# Autodesk Inventor assembly: Full Wheel
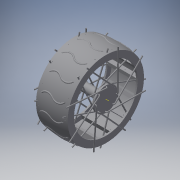
[picture p0: Inventor's stored thumbnail of the model, 180x180]
Saved by Autodesk Inventor 2019 (Build 230136000, 136)
## iProperties
Created: 2018-10-28
Part Number: Full Wheel
Document SubType Name: Assembly
Designer: Swapnil
Author: Swapnil
## Documents named in this file (3)
- C:\Users\Swapnil\Desktop\ImportantThings\Robotics\Vanderbilt Robotics\2018-2019\FrameAndDrive\Full Wheel.iam
- C:\Users\Swapnil\Desktop\ImportantThings\Robotics\Vanderbilt Robotics\2018-2019\FrameAndDrive\spoke hub with spokes.ipt
- C:\Users\Swapnil\Desktop\ImportantThings\Robotics\Vanderbilt Robotics\2018-2019\FrameAndDrive\Outerrim of the Wheel (new).ipt
## Components (2 placed, 2 different names)
1. spoke hub with spokes:1 — Mate:1, Flush:1
2. Outerrim of the Wheel (new):1 — Mate:1, Flush:1
## Relationships (2: Mate 1, Flush 1)
- Mate:1: spoke hub with spokes:1 ↔ Outerrim of the Wheel (new):1
- Flush:1: spoke hub with spokes:1 ↔ Outerrim of the Wheel (new):1
